# Autodesk Inventor assembly: Turnbuckle
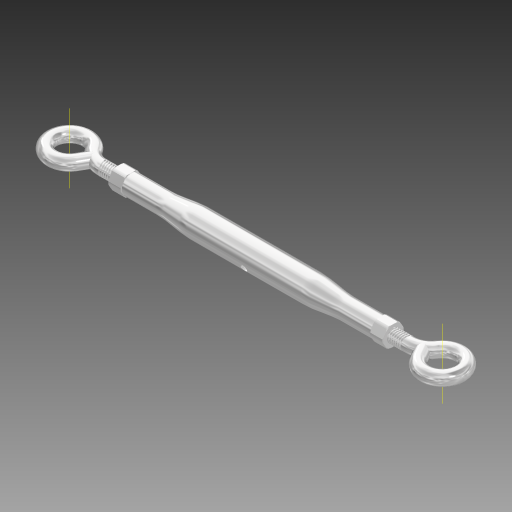
[picture p0: Inventor's stored thumbnail of the model, 512x512]
Saved by Autodesk Inventor 2023 (Build 270158030, 158C)
## iProperties
Created: 2023-01-25
Part Number: Turnbuckle
Document SubType Name: Assembly
Designer: Cal
Author: Cal
## Documents named in this file (3)
- D:\Collaborative Robots\COTS Parts\Elevators\COTS Parts\400Lb Capacity 6.5in Turnbuckle (McMaster 3082T11).iam
- D:\Collaborative Robots\COTS Parts\Elevators\COTS Parts\Base 400Lb Capacity 6.5in Turnbuckle (McMaster 3082T11).ipt
- D:\Collaborative Robots\COTS Parts\Elevators\COTS Parts\Arm 400Lb Capacity 6.5in Turnbuckle (McMaster 3082T11).ipt
## Components (3 placed, 2 different names)
1. Base 400Lb Capacity 6.5in Turnbuckle (McMaster 3082T11):1 — Insert:1, Insert:2, Mate:3, Flush:3
2. Arm 400Lb Capacity 6.5in Turnbuckle (McMaster 3082T11):1 — Insert:1, Flush:1, Mate:1, Flush:2, Symmetry:1
3. Arm 400Lb Capacity 6.5in Turnbuckle (McMaster 3082T11):2 — Insert:2, Flush:1, Mate:2, Symmetry:1
## Relationships (9: Flush 3, Mate 3, Insert 2, Symmetry 1)
- Insert:1: Base 400Lb Capacity 6.5in Turnbuckle (McMaster 3082T11):1 ↔ Arm 400Lb Capacity 6.5in Turnbuckle (McMaster 3082T11):1
- Insert:2: Base 400Lb Capacity 6.5in Turnbuckle (McMaster 3082T11):1 ↔ Arm 400Lb Capacity 6.5in Turnbuckle (McMaster 3082T11):2
- Flush:1: Arm 400Lb Capacity 6.5in Turnbuckle (McMaster 3082T11):1 ↔ Arm 400Lb Capacity 6.5in Turnbuckle (McMaster 3082T11):2
- Mate:1: Arm 400Lb Capacity 6.5in Turnbuckle (McMaster 3082T11):1
- Mate:2: Arm 400Lb Capacity 6.5in Turnbuckle (McMaster 3082T11):2
- Flush:2: Arm 400Lb Capacity 6.5in Turnbuckle (McMaster 3082T11):1
- Symmetry:1: Arm 400Lb Capacity 6.5in Turnbuckle (McMaster 3082T11):1 ↔ Arm 400Lb Capacity 6.5in Turnbuckle (McMaster 3082T11):2
- Mate:3: Base 400Lb Capacity 6.5in Turnbuckle (McMaster 3082T11):1
- Flush:3: Base 400Lb Capacity 6.5in Turnbuckle (McMaster 3082T11):1
